# Autodesk Inventor assembly: 50mmActuator
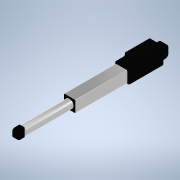
[picture p0: Inventor's stored thumbnail of the model, 180x180]
Saved by Autodesk Inventor 2020 (Build 240168000, 168)
## iProperties
Created: 2023-02-03
Part Number: 50mmActuator
Document SubType Name: Assembly
Designer: legoo
Author: legoo
## Documents named in this file (3)
- C:\Users\Public\Documents\Autodesk\Inventor 2020\projects\3156\actuators\50mm\50mmActuator.iam
- C:\Users\Public\Documents\Autodesk\Inventor 2020\projects\3156\actuators\50mm\50mmStrokeBase.ipt
- C:\Users\Public\Documents\Autodesk\Inventor 2020\projects\3156\actuators\50mm\50mmStrokeRod.ipt
## Components (2 placed, 2 different names)
1. 50mmStrokeBase:1 — Mate:1, Angle:1, Flush:1, Mate:2, Mate:3
2. 50mmStrokeRod:1 — Mate:1, Angle:1
## Relationships (5: Mate 3, Angle 1, Flush 1)
- Mate:1: 50mmStrokeBase:1 ↔ 50mmStrokeRod:1
- Angle:1 (0 deg): 50mmStrokeBase:1 ↔ 50mmStrokeRod:1
- Flush:1: 50mmStrokeBase:1
- Mate:2: 50mmStrokeBase:1
- Mate:3: 50mmStrokeBase:1
